# Autodesk Inventor assembly: Assembly Macaco
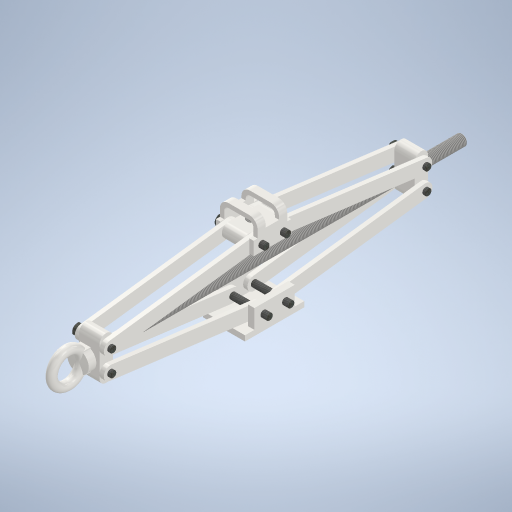
[picture p0: Inventor's stored thumbnail of the model, 512x512]
Saved by Autodesk Inventor 2024 (Build 280153000, 153)
## iProperties
Created: 2024-06-01
Part Number: Assembly Macaco
Document SubType Name: Assembly
Designer: Pedro
Mass: 6917.65 g
Surface Area: 2816.9 cm^2
Volume: 881.229 cm^3
Density: 7.85 g/cm^3
d10: 0,000 mm
w_Braço: 12,000 mm
Author: Pedro
## Documents named in this file (15)
- C:\Users\Pedro\Desktop\Autodesk Inbentor\Projeto\Assembly Macaco.iam
- C:\Users\Pedro\Desktop\Autodesk Inbentor\Projeto\Base Macaco.ipt
- C:\Users\Pedro\Desktop\Autodesk Inbentor\Projeto\Braço Macaco.ipt
- C:\Users\Pedro\Desktop\Autodesk Inbentor\Projeto\Junção Fuso.ipt
- C:\Users\Pedro\Desktop\Autodesk Inbentor\Projeto\Encaixe Macaco.ipt
- C:\Users\Pedro\Documents\Inventor\Content Center Files\R2024\en-US\ISO 4018\ISO 4018 - M12 x 80.ipt
- C:\Users\Pedro\Documents\Inventor\Content Center Files\R2024\en-US\ISO 4018\ISO 4018 - M12 x 60.ipt
- C:\Users\Pedro\Documents\Inventor\Content Center Files\R2024\en-US\ISO 4018\ISO 4018 - M12 x 90.ipt
- C:\Users\Pedro\Desktop\Autodesk Inbentor\Projeto\DIN 580 - M20 x 700 x 2,5 x 1,6.ipt
- C:\Users\Pedro\Desktop\Autodesk Inbentor\Projeto\Assembly Macaco\AIP\FEA\epzg9a0f4.fins
- C:\Users\Pedro\Desktop\Autodesk Inbentor\Projeto\Assembly Macaco\AIP\FEA\epzg9a0g0.fsat
- C:\Users\Pedro\Desktop\Autodesk Inbentor\Projeto\Assembly Macaco\AIP\FEA\epzg9a0g0.ftes
- C:\Users\Pedro\Desktop\Autodesk Inbentor\Projeto\Assembly Macaco\AIP\FEA\epzg9a0g0.fwiz
- C:\Users\Pedro\Desktop\Autodesk Inbentor\Projeto\Assembly Macaco\AIP\FEA\epzg9a0m8.fmsh
- C:\Users\Pedro\Desktop\Autodesk Inbentor\Projeto\Assembly Macaco\AIP\FEA\epzg9a0m9.fres
## Components (22 placed, 8 different names)
1. Base Macaco:1 — Insert:5, Insert:6, Insert:7, Angle:2, Angle:3, Mate:9, Insert:85, Insert:86
2. Braço Macaco:2 — Insert:5, Insert:9
3. Braço Macaco:3 — Insert:6, Insert:10, Insert:71, Insert:85
4. Braço Macaco:4 — Insert:7, Insert:73, Insert:83
5. Junção Fuso:1 — Insert:9, Insert:14, Insert:15, Angle:1, Mate:2, Insert:82, Insert:83
6. Junção Fuso:2 — Insert:10, Angle:1, Angle:2, Mate:2, Mate:6, Mate:10, Insert:81
7. Braço Macaco:5 — Insert:31, Mate:13
8. Braço Macaco:6 — Insert:14, Insert:32
9. Braço Macaco:7 — Mate:6, Insert:46, Insert:70, Insert:80
10. Braço Macaco:8 — Insert:15, Insert:72, Insert:84
11. Encaixe Macaco:1 — Insert:31, Insert:32, Angle:3, Insert:46, Mate:9, Insert:68, Insert:69, Insert:84
12. Braço Macaco:9 — Insert:81, Mate:12
13. ISO 4018 M12 x 80:1 — Insert:68
14. ISO 4018 M12 x 80:2 — Insert:69, Mate:11
15. ISO 4018 M12 x 60:1 — Insert:70, Mate:13
16. ISO 4018 M12 x 60:2 — Insert:71
17. ISO 4018 M12 x 60:3 — Insert:73
18. ISO 4018 M12 x 60:4 — Insert:72
19. ISO 4018 M12 x 90:1
20. ISO 4018 M12 x 90:2 — Mate:12, Insert:86
21. DIN 580 - M20 x 700 x 2,5 x 1,6:1 — Mate:10, Insert:82
22. Junção Fuso:3 — Insert:80, Mate:11
## Relationships (33: Insert 23, Mate 7, Angle 3)
- Insert:5: Base Macaco:1 ↔ Braço Macaco:2
- Insert:6: Base Macaco:1 ↔ Braço Macaco:3
- Insert:7: Base Macaco:1 ↔ Braço Macaco:4
- Insert:9: Braço Macaco:2 ↔ Junção Fuso:1
- Insert:10: Braço Macaco:3 ↔ Junção Fuso:2
- Insert:14: Junção Fuso:1 ↔ Braço Macaco:6
- Insert:15: Junção Fuso:1 ↔ Braço Macaco:8
- Insert:31: Braço Macaco:5 ↔ Encaixe Macaco:1
- Insert:32: Braço Macaco:6 ↔ Encaixe Macaco:1
- Angle:1 (180 deg): Junção Fuso:1 ↔ Junção Fuso:2
- Angle:2 (0 deg): Base Macaco:1 ↔ Junção Fuso:2
- Mate:2 (252.272 mm): Junção Fuso:1 ↔ Junção Fuso:2
- Mate:6: Junção Fuso:2 ↔ Braço Macaco:7
- Angle:3 (180 deg): Base Macaco:1 ↔ Encaixe Macaco:1
- Insert:46: Braço Macaco:7 ↔ Encaixe Macaco:1
- Mate:9 (174.827 mm): Base Macaco:1 ↔ Encaixe Macaco:1
- Insert:68: Encaixe Macaco:1 ↔ ISO 4018 M12 x 80:1
- Insert:69: Encaixe Macaco:1 ↔ ISO 4018 M12 x 80:2
- Insert:70: Braço Macaco:7 ↔ ISO 4018 M12 x 60:1
- Insert:71: Braço Macaco:3 ↔ ISO 4018 M12 x 60:2
- Insert:72: Braço Macaco:8 ↔ ISO 4018 M12 x 60:4
- Insert:73: Braço Macaco:4 ↔ ISO 4018 M12 x 60:3
- Mate:10: Junção Fuso:2 ↔ DIN 580 - M20 x 700 x 2,5 x 1,6:1
- Insert:80: Braço Macaco:7 ↔ Junção Fuso:3
- Mate:11: ISO 4018 M12 x 80:2 ↔ Junção Fuso:3
- Insert:81: Junção Fuso:2 ↔ Braço Macaco:9
- Mate:12: Braço Macaco:9 ↔ ISO 4018 M12 x 90:2
- Insert:82: Junção Fuso:1 ↔ DIN 580 - M20 x 700 x 2,5 x 1,6:1
- Mate:13: Braço Macaco:5 ↔ ISO 4018 M12 x 60:1
- Insert:83: Braço Macaco:4 ↔ Junção Fuso:1
- Insert:84: Braço Macaco:8 ↔ Encaixe Macaco:1
- Insert:85: Base Macaco:1 ↔ Braço Macaco:3
- Insert:86: Base Macaco:1 ↔ ISO 4018 M12 x 90:2
## Named parameters: sa_0 = 981000, sa_1 = 981000
note: some values were not read from the file. Shown as the stored number, unit unknown: "sa_0", "sa_1".
